# Autodesk Inventor assembly: Сборка5
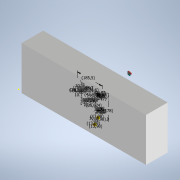
[picture p0: Inventor's stored thumbnail of the model, 180x180]
Saved by Autodesk Inventor 2022 (Build 260153000, 153)
## iProperties
Created: 2022-07-29
Part Number: Сборка5
Document SubType Name: Assembly
Designer: akapu
Author: akapu
## Documents named in this file (48)
- C:\Users\akapu\OneDrive\Документы\maze bot\Сборка5.iam
- C:\Users\akapu\OneDrive\Документы\maze bot\maze_04.ipt
- C:\Users\akapu\OneDrive\Документы\maze bot\motor.ipt
- C:\Users\akapu\OneDrive\Документы\maze bot\motor_ЗЕРКАЛО.ipt
- C:\Users\akapu\OneDrive\Документы\maze bot\akkum_holder_up.ipt
- C:\Users\akapu\OneDrive\Документы\maze bot\akkum_holder.ipt
- C:\Users\akapu\OneDrive\Документы\maze bot\metal_holder.ipt
- C:\Users\akapu\OneDrive\Документы\maze bot\rama.ipt
- C:\Users\akapu\OneDrive\Документы\maze bot\vydacha_4.ipt
- C:\Users\akapu\OneDrive\Документы\maze bot\pizza.ipt
- C:\Users\akapu\OneDrive\Документы\maze bot\pizza_disk.ipt
- C:\Users\akapu\OneDrive\Документы\maze bot\pizza_2.ipt
- C:\Users\akapu\OneDrive\Документы\maze bot\mg996r v17.iam
- C:\Users\akapu\OneDrive\Документы\maze bot\reyka_3.ipt
- C:\Users\akapu\OneDrive\Документы\maze bot\lid.ipt
- C:\Users\akapu\OneDrive\Документы\maze bot\vagonetka_2.ipt
- C:\Users\akapu\OneDrive\Документы\maze bot\wheel_5.ipt
- C:\Users\akapu\OneDrive\Документы\maze bot\block.ipt
- C:\Users\akapu\OneDrive\Документы\maze bot\rolik_2.ipt
- C:\Users\akapu\OneDrive\Документы\maze bot\защёлка_выдача2.ipt
- C:\Users\akapu\OneDrive\Документы\maze bot\держатель_гаек.ipt
- C:\Users\akapu\OneDrive\Документы\maze bot\разделитель.ipt
- C:\Users\akapu\OneDrive\Документы\maze bot\block_01.ipt
- C:\Users\akapu\OneDrive\Документы\maze bot\block_02.ipt
- C:\Users\akapu\OneDrive\Документы\maze bot\lab.ipt
- C:\Users\akapu\OneDrive\Документы\maze bot\victum.ipt
- C:\Users\akapu\OneDrive\Документы\maze bot\cameraFOV.ipt
- C:\Users\akapu\OneDrive\Документы\maze bot\view_centre.ipt
- C:\Users\akapu\OneDrive\Документы\maze bot\OpenMV H7\openmv4_h7.iam
- C:\Users\akapu\OneDrive\Документы\maze bot\vision.ipt
- C:\Users\akapu\OneDrive\Документы\maze bot\vision_centre.ipt
- C:\Users\akapu\OneDrive\Документы\projects_xz\temp.ipt
- C:\Users\akapu\OneDrive\Документы\maze bot\temp_vision.ipt
- C:\Users\akapu\OneDrive\Документы\maze bot\OpenMV H7\openmv4_h7_base_® ã¬®«ç ­¨î.iam
- C:\Users\akapu\OneDrive\Документы\maze bot\end_cap.ipt
- C:\Users\akapu\OneDrive\Документы\maze bot\cap_end_cap.ipt
- C:\Users\akapu\OneDrive\Документы\maze bot\end cap left.ipt
- C:\Users\akapu\OneDrive\Документы\maze bot\end cap right.ipt
- C:\Users\akapu\OneDrive\Документы\maze bot\cap_end_cap_left.ipt
- C:\Users\akapu\OneDrive\Документы\maze bot\vl53l0x\vl53l0x_PCB.ipt
- C:\Users\akapu\OneDrive\Документы\maze bot\button_krepl.ipt
- C:\Users\akapu\OneDrive\Документы\maze bot\fast_akkum2.iam
- C:\Users\akapu\OneDrive\Документы\maze bot\lazer_side.ipt
- C:\Users\akapu\OneDrive\Документы\maze bot\laser_krepl.ipt
- C:\Users\akapu\OneDrive\Документы\maze bot\Motherboard.ipt
- C:\Users\akapu\OneDrive\Документы\maze bot\laser_krepl_2.ipt
- C:\Users\akapu\OneDrive\Документы\maze bot\laser_krepl_right.ipt
- C:\Users\akapu\OneDrive\Документы\maze bot\cherrry red\cherry mx.ipt
## Components (65 placed, 47 different names)
1. maze_04:1 — С поворотом:1, С поворотом:2, С поворотом:3, С поворотом:4, Вставка:1, Вставка:4, С поворотом:5, Совмещение:7, Совмещение:8, Совмещение:9, Совмещение:11, Совмещение:12, Совмещение:13, Совмещение:27, Совмещение:31, Совмещение:32, Совмещение:33, Совмещение:34, Совмещение:35, Совмещение:36, Совмещение:37, Совмещение:52, Совмещение:53, Совмещение:54, Совмещение:59, Заподлицо:63, Заподлицо:64, Жесткий:1, Совмещение:149, С поворотом:18, С поворотом:19, С поворотом:26, С поворотом:27
2. motor:1 — С поворотом:1, Совмещение:12, Вставка:6, Совмещение:29
3. motor:2 — С поворотом:2, Совмещение:8, Вставка:8, Совмещение:28
4. motor_ЗЕРКАЛО:1 — С поворотом:3, Совмещение:7, Вставка:7, Совмещение:26
5. motor_ЗЕРКАЛО:2 — С поворотом:4, Совмещение:9, Совмещение:10, Совмещение:11, Вставка:9, Совмещение:30
6. akkum_holder_up:1 — Вставка:1, Совмещение:13, Flush:66, Совмещение:153, Совмещение:154, Совмещение:155
7. akkum_holder:1 — Жесткий:1, Жесткий:2
8. metal_holder:1 — Жесткий:2
9. rama:1 — Вставка:4, С поворотом:5, С поворотом:6, Совмещение:48, С поворотом:9, Совмещение:55, Шаровой:3, Совмещение:67, Жесткий:12, С поворотом:28, С поворотом:29, Совмещение:159, Совмещение:160, Совмещение:161
10. vydacha_4:1 — С поворотом:6, Совмещение:10, Заподлицо:73
11. pizza:1 — Совмещение:2, Совмещение:3, С поворотом:8, Совмещение:19, Угол:2, Совмещение:49, С поворотом:9, Совмещение:55
12. pizza_disk:1 — Совмещение:2, Совмещение:3, Угол:2, Совмещение:56
13. pizza_2:1 — Совмещение:48, Совмещение:49, Совмещение:56
14. mg996r v17:1 [sub-assembly]
15. reyka_3:1 — С поворотом:8, Совмещение:19, Вставка:5, Совмещение:20, Совмещение:21, Угол:1, Совмещение:42, Заподлицо:67, Заподлицо:74, Заподлицо:75, Заподлицо:77
16. lid:1 — Вставка:5, Совмещение:23, Совмещение:24, Совмещение:25, Совмещение:39, Совмещение:40, Совмещение:41, Угол:1, Совмещение:43, Совмещение:50
17. vagonetka_2:1 — Совмещение:20, Совмещение:21, Совмещение:42
18. wheel_5:1 — Вставка:6
19. wheel_5:2 — Вставка:7
20. wheel_5:3 — Вставка:9
21. wheel_5:4 — Вставка:8
22. block:1
23. rolik_2:1 — Совмещение:43, Совмещение:50
24. защёлка_выдача2:1 — Совмещение:23, Совмещение:24, Совмещение:25
25. держатель_гаек:1 — Совмещение:26, Совмещение:27, Совмещение:35
26. держатель_гаек:2 — Совмещение:28, Совмещение:32, Совмещение:34
27. держатель_гаек:3 — Совмещение:29, Совмещение:33, Совмещение:36
28. держатель_гаек:4 — Совмещение:30, Совмещение:31, Совмещение:37
29. разделитель:1 — Совмещение:39, Совмещение:40, Совмещение:41
30. block_01:1 — Вставка:11
31. block_02:1 — Вставка:11
32. lab:1 — Совмещение:52, Совмещение:53, Совмещение:54, Заподлицо:58, Совмещение:57, Заподлицо:59, Заподлицо:60, Совмещение:58
33. victum:1 — Заподлицо:59, Заподлицо:60, Совмещение:58, Совмещение:59, Шаровой:5
34. cameraFOV:1 — Заподлицо:61, Совмещение:65, Заподлицо:62, Шаровой:2, Совмещение:69
35. view_centre:1 — Шаровой:5, Совмещение:69
36. openmv4_h7_base_® ã¬®«ç ­¨î_1 [sub-assembly] — Flush:66
37. openmv4_h7:1 [sub-assembly] — Заподлицо:61, Совмещение:65, Заподлицо:62, Совмещение:149, Заподлицо:67
38. vision:1 — Шаровой:2, Совмещение:66, Совмещение:68
39. vision_centre:1 — Шаровой:3, Совмещение:66
40. vision_centre:2 — Шаровой:4, Совмещение:67
41. vision_centre:3 — Шаровой:4, Совмещение:68
42. temp_level:1 — Заподлицо:63, Заподлицо:64
43. temp_vision:1
44. end_cap:1 — С поворотом:11
45. end_cap:2 — С поворотом:10
46. cap_end_cap:1
47. end cap left:1 — Жесткий:12, Совмещение:146, Совмещение:147, Совмещение:148, С поворотом:10
48. end cap right:1 — С поворотом:11, С поворотом:28, С поворотом:29
49. cap_end_cap_left:1 — Совмещение:146, Совмещение:147, Совмещение:148
50. vl53l0x_PCB:1 — С поворотом:20, С поворотом:21
51. vl53l0x_PCB:3 — С поворотом:24, С поворотом:25
52. vl53l0x_PCB:4 — С поворотом:22, С поворотом:23
53. vl53l0x_PCB:5
54. vl53l0x_PCB:6
55. button_krepl:1 — Заподлицо:73
56. fast_akkum2:1 [sub-assembly] — Совмещение:153, Совмещение:154, Совмещение:155
57. lazer_side:1 — С поворотом:18, С поворотом:19, С поворотом:20, С поворотом:21
58. lazer_side:2 — С поворотом:24, С поворотом:25, С поворотом:26, С поворотом:27
59. lazer_side:3 — С поворотом:22, С поворотом:23
60. laser_krepl:1 — Заподлицо:74, Заподлицо:76, С поворотом:30, С поворотом:31
61. Motherboard:1 — Совмещение:159, Совмещение:160, Совмещение:161
62. laser_krepl_2:1 — Заподлицо:75, Заподлицо:76, С поворотом:30, С поворотом:31
63. laser_krepl_right:1 — Заподлицо:77
64. cherry mx:1
65. cherry mx:2
## Relationships (113: Mate 58, RevoluteJoint 24, Flush 14, Insert 8, BallJoint 4, WeldJoint 3, Angle 2)
- С поворотом:1 [RevoluteJoint]: maze_04:1 ↔ motor:1
- С поворотом:2 [RevoluteJoint]: maze_04:1 ↔ motor:2
- С поворотом:3 [RevoluteJoint]: maze_04:1 ↔ motor_ЗЕРКАЛО:1
- С поворотом:4 [RevoluteJoint]: maze_04:1 ↔ motor_ЗЕРКАЛО:2
- Вставка:1 [Insert]: maze_04:1 ↔ akkum_holder_up:1
- Вставка:4 [Insert]: maze_04:1 ↔ rama:1
- С поворотом:5 [RevoluteJoint]: maze_04:1 ↔ rama:1
- С поворотом:6 [RevoluteJoint]: rama:1 ↔ vydacha_4:1
- Совмещение:2 [Mate]: pizza:1 ↔ pizza_disk:1
- Совмещение:3 [Mate]: pizza:1 ↔ pizza_disk:1
- Совмещение:7 [Mate]: maze_04:1 ↔ motor_ЗЕРКАЛО:1
- Совмещение:8 [Mate]: maze_04:1 ↔ motor:2
- Совмещение:9 [Mate]: maze_04:1 ↔ motor_ЗЕРКАЛО:2
- Совмещение:10 [Mate]: motor_ЗЕРКАЛО:2 ↔ vydacha_4:1
- Совмещение:11 [Mate]: maze_04:1 ↔ motor_ЗЕРКАЛО:2
- Совмещение:12 [Mate]: maze_04:1 ↔ motor:1
- Совмещение:13 [Mate]: maze_04:1 ↔ akkum_holder_up:1
- С поворотом:8 [RevoluteJoint]: pizza:1 ↔ reyka_3:1
- Совмещение:19 [Mate]: pizza:1 ↔ reyka_3:1
- Вставка:5 [Insert] (0.5 mm): reyka_3:1 ↔ lid:1
- Совмещение:20 [Mate]: reyka_3:1 ↔ vagonetka_2:1
- Совмещение:21 [Mate]: reyka_3:1 ↔ vagonetka_2:1
- Вставка:6 [Insert]: motor:1 ↔ wheel_5:1
- Вставка:7 [Insert]: motor_ЗЕРКАЛО:1 ↔ wheel_5:2
- Вставка:8 [Insert]: motor:2 ↔ wheel_5:4
- Вставка:9 [Insert]: motor_ЗЕРКАЛО:2 ↔ wheel_5:3
- Совмещение:23 [Mate]: lid:1 ↔ защёлка_выдача2:1
- Совмещение:24 [Mate] (-5.2 mm): lid:1 ↔ защёлка_выдача2:1
- Совмещение:25 [Mate]: lid:1 ↔ защёлка_выдача2:1
- Совмещение:26 [Mate]: motor_ЗЕРКАЛО:1 ↔ держатель_гаек:1
- Совмещение:27 [Mate]: maze_04:1 ↔ держатель_гаек:1
- Совмещение:28 [Mate]: motor:2 ↔ держатель_гаек:2
- Совмещение:29 [Mate]: motor:1 ↔ держатель_гаек:3
- Совмещение:30 [Mate]: motor_ЗЕРКАЛО:2 ↔ держатель_гаек:4
- Совмещение:31 [Mate]: maze_04:1 ↔ держатель_гаек:4
- Совмещение:32 [Mate]: maze_04:1 ↔ держатель_гаек:2
- Совмещение:33 [Mate]: maze_04:1 ↔ держатель_гаек:3
- Совмещение:34 [Mate]: maze_04:1 ↔ держатель_гаек:2
- Совмещение:35 [Mate]: maze_04:1 ↔ держатель_гаек:1
- Совмещение:36 [Mate]: maze_04:1 ↔ держатель_гаек:3
- Совмещение:37 [Mate]: maze_04:1 ↔ держатель_гаек:4
- Совмещение:39 [Mate]: lid:1 ↔ разделитель:1
- Совмещение:40 [Mate]: lid:1 ↔ разделитель:1
- Совмещение:41 [Mate]: lid:1 ↔ разделитель:1
- Угол:1 [Angle] (0 deg): reyka_3:1 ↔ lid:1
- Угол:2 [Angle] (0 deg): pizza:1 ↔ pizza_disk:1
- Совмещение:42 [Mate]: reyka_3:1 ↔ vagonetka_2:1
- Вставка:11 [Insert] (-3 mm): block_01:1 ↔ block_02:1
- Совмещение:43 [Mate]: lid:1 ↔ rolik_2:1
- Совмещение:48 [Mate] (-3 mm): rama:1 ↔ pizza_2:1
- Совмещение:49 [Mate]: pizza:1 ↔ pizza_2:1
- Совмещение:50 [Mate]: lid:1 ↔ rolik_2:1
- Совмещение:52 [Mate]: maze_04:1 ↔ lab:1
- Совмещение:53 [Mate] (66 mm): maze_04:1 ↔ lab:1
- Совмещение:54 [Mate]: maze_04:1 ↔ lab:1
- С поворотом:9 [RevoluteJoint]: rama:1 ↔ pizza:1
- Совмещение:55 [Mate]: rama:1 ↔ pizza:1
- Совмещение:56 [Mate]: pizza_disk:1 ↔ pizza_2:1
- Заподлицо:58 [Flush]: lab:1
- Совмещение:57 [Mate]: lab:1
- Заподлицо:59 [Flush]: lab:1 ↔ victum:1
- Заподлицо:60 [Flush]: lab:1 ↔ victum:1
- Совмещение:58 [Mate]: lab:1 ↔ victum:1
- Совмещение:59 [Mate]: maze_04:1 ↔ victum:1
- Заподлицо:61 [Flush] (29.453 mm): cameraFOV:1 ↔ openmv4_h7:1
- Совмещение:65 [Mate]: cameraFOV:1 ↔ openmv4_h7:1
- Заподлицо:62 [Flush]: cameraFOV:1 ↔ openmv4_h7:1
- Шаровой:2 [BallJoint]: cameraFOV:1 ↔ vision:1
- Шаровой:3 [BallJoint]: rama:1 ↔ vision_centre:1
- Совмещение:66 [Mate]: vision:1 ↔ vision_centre:1
- Шаровой:4 [BallJoint]: vision_centre:2 ↔ vision_centre:3
- Совмещение:67 [Mate]: rama:1 ↔ vision_centre:2
- Совмещение:68 [Mate]: vision:1 ↔ vision_centre:3
- Шаровой:5 [BallJoint]: victum:1 ↔ view_centre:1
- Совмещение:69 [Mate]: cameraFOV:1 ↔ view_centre:1
- Заподлицо:63 [Flush]: maze_04:1 ↔ temp_level:1
- Заподлицо:64 [Flush] (14 mm): maze_04:1 ↔ temp_level:1
- Flush:66: akkum_holder_up:1 ↔ openmv4_h7_base_® ã¬®«ç ­¨î_1
- Жесткий:1 [WeldJoint]: maze_04:1 ↔ akkum_holder:1
- Жесткий:2 [WeldJoint]: akkum_holder:1 ↔ metal_holder:1
- Жесткий:12 [WeldJoint]: rama:1 ↔ end cap left:1
- Совмещение:146 [Mate]: end cap left:1 ↔ cap_end_cap_left:1
- Совмещение:147 [Mate]: end cap left:1 ↔ cap_end_cap_left:1
- Совмещение:148 [Mate]: end cap left:1 ↔ cap_end_cap_left:1
- С поворотом:10 [RevoluteJoint]: end_cap:2 ↔ end cap left:1
- С поворотом:11 [RevoluteJoint]: end_cap:1 ↔ end cap right:1
- Совмещение:149 [Mate]: maze_04:1 ↔ openmv4_h7:1
- Заподлицо:67 [Flush]: reyka_3:1 ↔ openmv4_h7:1
- Заподлицо:73 [Flush]: vydacha_4:1 ↔ button_krepl:1
- Совмещение:153 [Mate]: akkum_holder_up:1 ↔ fast_akkum2:1
- Совмещение:154 [Mate]: akkum_holder_up:1 ↔ fast_akkum2:1
- Совмещение:155 [Mate]: akkum_holder_up:1 ↔ fast_akkum2:1
- С поворотом:18 [RevoluteJoint]: maze_04:1 ↔ lazer_side:1
- С поворотом:19 [RevoluteJoint]: maze_04:1 ↔ lazer_side:1
- С поворотом:20 [RevoluteJoint]: vl53l0x_PCB:1 ↔ lazer_side:1
- С поворотом:21 [RevoluteJoint]: vl53l0x_PCB:1 ↔ lazer_side:1
- С поворотом:22 [RevoluteJoint]: vl53l0x_PCB:4 ↔ lazer_side:3
- С поворотом:23 [RevoluteJoint]: vl53l0x_PCB:4 ↔ lazer_side:3
- С поворотом:24 [RevoluteJoint]: vl53l0x_PCB:3 ↔ lazer_side:2
- С поворотом:25 [RevoluteJoint]: vl53l0x_PCB:3 ↔ lazer_side:2
- С поворотом:26 [RevoluteJoint]: maze_04:1 ↔ lazer_side:2
- С поворотом:27 [RevoluteJoint]: maze_04:1 ↔ lazer_side:2
- С поворотом:28 [RevoluteJoint]: rama:1 ↔ end cap right:1
- С поворотом:29 [RevoluteJoint]: rama:1 ↔ end cap right:1
- Заподлицо:74 [Flush]: reyka_3:1 ↔ laser_krepl:1
- Совмещение:159 [Mate]: rama:1 ↔ Motherboard:1
- Совмещение:160 [Mate]: rama:1 ↔ Motherboard:1
- Совмещение:161 [Mate] (11 mm): rama:1 ↔ Motherboard:1
- Заподлицо:75 [Flush]: reyka_3:1 ↔ laser_krepl_2:1
- Заподлицо:76 [Flush]: laser_krepl:1 ↔ laser_krepl_2:1
- С поворотом:30 [RevoluteJoint]: laser_krepl:1 ↔ laser_krepl_2:1
- С поворотом:31 [RevoluteJoint]: laser_krepl:1 ↔ laser_krepl_2:1
- Заподлицо:77 [Flush]: reyka_3:1 ↔ laser_krepl_right:1
